# Autodesk Inventor assembly: bottom cover assy
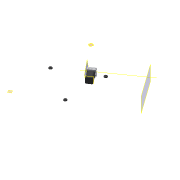
[picture p0: Inventor's stored thumbnail of the model, 180x180]
Saved by Autodesk Inventor 2016 (Build 200138000, 138)
## iProperties
Created: 2016-08-18
Part Number: bottom cover assy
Document SubType Name: Assembly
Designer: admin
Author: admin
## Documents named in this file (19)
- C:\Users\Juny\OneDrive - (주)에이팀벤처스\ateam\CL 3D프린터 사업- 설계 이준영\(((( delta 3D printer))))\20. 20190104 D3\1612 D3 3D modeling\bottom cover assy\bottom cover assy.iam
- C:\Users\Juny\OneDrive - (주)에이팀벤처스\ateam\CL 3D프린터 사업- 설계 이준영\(((( delta 3D printer))))\20. 20190104 D3\1612 D3 3D modeling\bottom cover assy\bearing.ipt
- C:\Users\Juny\OneDrive - (주)에이팀벤처스\ateam\CL 3D프린터 사업- 설계 이준영\(((( delta 3D printer))))\20. 20190104 D3\1612 D3 3D modeling\bottom cover assy\clamp_fixer.ipt
- C:\Users\Juny\OneDrive - (주)에이팀벤처스\ateam\CL 3D프린터 사업- 설계 이준영\(((( delta 3D printer))))\20. 20190104 D3\1612 D3 3D modeling\bottom cover assy\feeder botton new.ipt
- C:\Users\Juny\OneDrive - (주)에이팀벤처스\ateam\CL 3D프린터 사업- 설계 이준영\(((( delta 3D printer))))\20. 20190104 D3\1612 D3 3D modeling\bottom cover assy\feeder laver new.ipt
- C:\Users\Juny\OneDrive - (주)에이팀벤처스\ateam\CL 3D프린터 사업- 설계 이준영\(((( delta 3D printer))))\20. 20190104 D3\1612 D3 3D modeling\bottom cover assy\feeder top new.ipt
- C:\Users\Juny\OneDrive - (주)에이팀벤처스\ateam\CL 3D프린터 사업- 설계 이준영\(((( delta 3D printer))))\20. 20190104 D3\1612 D3 3D modeling\bottom cover assy\m3 25 socket_screw.ipt
- C:\Users\Juny\OneDrive - (주)에이팀벤처스\ateam\CL 3D프린터 사업- 설계 이준영\(((( delta 3D printer))))\20. 20190104 D3\1612 D3 3D modeling\bottom cover assy\m3 sqaure nut.ipt
- C:\Users\Juny\OneDrive - (주)에이팀벤처스\ateam\CL 3D프린터 사업- 설계 이준영\(((( delta 3D printer))))\20. 20190104 D3\1612 D3 3D modeling\bottom cover assy\M5 25 button head.ipt
- C:\Users\Juny\OneDrive - (주)에이팀벤처스\ateam\CL 3D프린터 사업- 설계 이준영\(((( delta 3D printer))))\20. 20190104 D3\1612 D3 3D modeling\bottom cover assy\M5_square_nut.ipt
- C:\Users\Juny\OneDrive - (주)에이팀벤처스\ateam\CL 3D프린터 사업- 설계 이준영\(((( delta 3D printer))))\20. 20190104 D3\1612 D3 3D modeling\bottom cover assy\nut_M4.ipt
- C:\Users\Juny\OneDrive - (주)에이팀벤처스\ateam\CL 3D프린터 사업- 설계 이준영\(((( delta 3D printer))))\20. 20190104 D3\1612 D3 3D modeling\bottom cover assy\pinion_gear.ipt
- C:\Users\Juny\OneDrive - (주)에이팀벤처스\ateam\CL 3D프린터 사업- 설계 이준영\(((( delta 3D printer))))\20. 20190104 D3\1612 D3 3D modeling\bottom cover assy\rubber_foot.ipt
- C:\Users\Juny\OneDrive - (주)에이팀벤처스\ateam\CL 3D프린터 사업- 설계 이준영\(((( delta 3D printer))))\20. 20190104 D3\1612 D3 3D modeling\bottom cover assy\spring.ipt
- C:\Users\Juny\OneDrive - (주)에이팀벤처스\ateam\CL 3D프린터 사업- 설계 이준영\(((( delta 3D printer))))\20. 20190104 D3\1612 D3 3D modeling\bottom cover assy\stepping_motor f.ipt
- C:\Users\Juny\OneDrive - (주)에이팀벤처스\ateam\CL 3D프린터 사업- 설계 이준영\(((( delta 3D printer))))\20. 20190104 D3\1612 D3 3D modeling\bottom cover assy\tube clamp.ipt
- C:\Users\Juny\OneDrive - (주)에이팀벤처스\ateam\CL 3D프린터 사업- 설계 이준영\(((( delta 3D printer))))\20. 20190104 D3\1612 D3 3D modeling\bottom cover assy\tubeclamp male.ipt
- C:\Users\Juny\OneDrive - (주)에이팀벤처스\ateam\CL 3D프린터 사업- 설계 이준영\(((( delta 3D printer))))\20. 20190104 D3\1612 D3 3D modeling\bottom cover assy\m4 12 Button Head.ipt
- C:\Users\Juny\OneDrive - (주)에이팀벤처스\ateam\CL 3D프린터 사업- 설계 이준영\(((( delta 3D printer))))\20. 20190104 D3\1612 D3 3D modeling\bottom cover assy\m3 15 socket_screw.ipt
## Components (21 placed, 18 different names)
1. bearing:1 — Rotational:4
2. clamp_fixer:1 — Rotational:19
3. feeder botton new:1 — Rotational:2, Mate:1, Rotational:8, Cylindrical:1, Rotational:10, Rotational:13, Angle:2, Rotational:17
4. feeder laver new:1 — Rotational:4, Rotational:5, Rotational:6, Mate:1, Angle:1, Mate:2
5. feeder top new:1 — Rotational:8, Cylindrical:1, Rotational:9, Rotational:11, Rotational:12, Mate:2
6. m3 25 socket_screw:1 — Rotational:12
7. m3 sqaure nut:1 — Rotational:10
8. M5 25 button head:1 — Rotational:1, Rotational:2, Angle:1
9. M5_square_nut:1 — Rotational:1, Rotational:7
10. nut_M4:1 — Rotational:6
11. pinion_gear:1 — Rotational:3
12. rubber_foot:1
13. spring:1 — Rotational:7
14. stepping_motor f:1 — Rotational:3, Rotational:13, Angle:2
15. tube clamp:1 — Rotational:17, Rotational:18, Rotational:19
16. tubeclamp male:1 — Rotational:18
17. m4 12 Button Head:1 — Rotational:5
18. m3 25 socket_screw:2 — Rotational:11
19. m3 15 socket_screw:1 — Rotational:9
20. rubber_foot:2
21. rubber_foot:3
## Relationships (21: RevoluteJoint 16, Mate 2, Angle 2, CylindricalJoint 1)
- Rotational:1 [RevoluteJoint] (-7 mm): M5 25 button head:1 ↔ M5_square_nut:1
- Rotational:2 [RevoluteJoint]: feeder botton new:1 ↔ M5 25 button head:1
- Rotational:3 [RevoluteJoint] (-4 mm): pinion_gear:1 ↔ stepping_motor f:1
- Rotational:4 [RevoluteJoint] (0.2 mm): bearing:1 ↔ feeder laver new:1
- Rotational:5 [RevoluteJoint]: feeder laver new:1 ↔ m4 12 Button Head:1
- Rotational:6 [RevoluteJoint]: feeder laver new:1 ↔ nut_M4:1
- Mate:1: feeder botton new:1 ↔ feeder laver new:1
- Angle:1 (0 deg): feeder laver new:1 ↔ M5 25 button head:1
- Rotational:7 [RevoluteJoint]: M5_square_nut:1 ↔ spring:1
- Rotational:8 [RevoluteJoint]: feeder botton new:1 ↔ feeder top new:1
- Cylindrical:1: feeder botton new:1 ↔ feeder top new:1
- Rotational:9 [RevoluteJoint]: feeder top new:1 ↔ m3 15 socket_screw:1
- Rotational:10 [RevoluteJoint]: feeder botton new:1 ↔ m3 sqaure nut:1
- Rotational:11 [RevoluteJoint]: feeder top new:1 ↔ m3 25 socket_screw:2
- Rotational:12 [RevoluteJoint]: feeder top new:1 ↔ m3 25 socket_screw:1
- Mate:2 (0.2 mm): feeder laver new:1 ↔ feeder top new:1
- Rotational:13 [RevoluteJoint] (3 mm): feeder botton new:1 ↔ stepping_motor f:1
- Angle:2 (0 deg): feeder botton new:1 ↔ stepping_motor f:1
- Rotational:17 [RevoluteJoint]: feeder botton new:1 ↔ tube clamp:1
- Rotational:18 [RevoluteJoint] (-1 mm): tube clamp:1 ↔ tubeclamp male:1
- Rotational:19 [RevoluteJoint]: clamp_fixer:1 ↔ tube clamp:1
